# Autodesk Inventor assembly: Bearing mounting assembly.SLDPRT
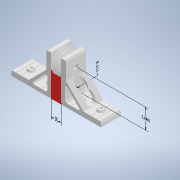
[picture p0: Inventor's stored thumbnail of the model, 180x180]
Saved by Autodesk Inventor 2020.2 (Build 242310000, 310)
## iProperties
Created: 2018-01-10
Part Number: Bearing mounting assembly.SLDPRT
Document SubType Name: Assembly
Designer: robst
Author: robst
Revision Number: ANY
## Documents named in this file (7)
- C:\git\CAD-Development\robSteele\2020LiftMechanism\Bearing mounting assembly.SLDPRT.iam
- C:\git\CAD-Development\robSteele\2020LiftMechanism\REV-21-1203 Preload 2 Screws Assembly.iam
- C:\git\CAD-Development\robSteele\2020LiftMechanism\10-32 Slim Nylock Nut.ipt
- C:\git\CAD-Development\robSteele\2020LiftMechanism\Bearing Delrin Spacer.ipt
- C:\git\CAD-Development\robSteele\2020LiftMechanism\REV-29-1014.ipt
- C:\git\CAD-Development\robSteele\2020LiftMechanism\10-32 1.5 inch Long.ipt
- C:\git\CAD-Development\robSteele\2020LiftMechanism\preventWireJumping.ipt
## Components (7 placed, 7 different names)
1. REV-21-1203 Preload 2 Screws Assembly_64 [sub-assembly]
2. REV-21-1203 Preload 2 Screws Assembly_65 [sub-assembly] — Insert:1, Flush:1
3. 10-32 Slim Nylock Nut_66
4. Bearing Delrin Spacer_67
5. REV-29-1014_68
6. 10-32 1.5 inch Long_69
7. preventWireJumping:1 — Insert:1, Flush:1
## Relationships (2: Insert 1, Flush 1)
- Insert:1: REV-21-1203 Preload 2 Screws Assembly_65 ↔ preventWireJumping:1
- Flush:1: REV-21-1203 Preload 2 Screws Assembly_65 ↔ preventWireJumping:1
